# Autodesk Inventor assembly: Backpack
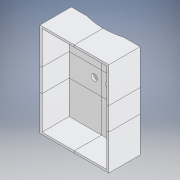
[picture p0: Inventor's stored thumbnail of the model, 180x180]
Saved by Autodesk Inventor 2017 SP1 (Build 210196100, 196)
## iProperties
Created: 2017-09-05
Part Number: Backpack
Document SubType Name: Assembly
Designer: Zach
Author: Zach
## Documents named in this file (8)
- C:\Users\Zach\Documents\GitHub\tr1\src\Body\Chest Assembly\Backpack Assembly\Backpack.iam
- C:\Users\Zach\Documents\GitHub\tr1\src\Body\Chest Assembly\Backpack Assembly\BP001.ipt
- C:\Users\Zach\Documents\GitHub\tr1\src\Body\Chest Assembly\Backpack Assembly\BP002.ipt
- C:\Users\Zach\Documents\GitHub\tr1\src\Body\Chest Assembly\Backpack Assembly\BP003.ipt
- C:\Users\Zach\Documents\GitHub\tr1\src\Body\Chest Assembly\Backpack Assembly\BP004.ipt
- C:\Users\Zach\Documents\GitHub\tr1\src\Body\Chest Assembly\Backpack Assembly\BP005.ipt
- C:\Users\Zach\Documents\GitHub\tr1\src\Body\Chest Assembly\Backpack Assembly\Ethernet Port.ipt
- C:\Users\Zach\Documents\GitHub\tr1\src\Body\Chest Assembly\Backpack Assembly\USB Hub.ipt
## Components (8 placed, 7 different names)
1. BP001:1 — Mate:1, Mate:2, Mate:3, Mate:4, Flush:1, Flush:3, Flush:7, Flush:12, Mate:16, Flush:15, Mate:17, Mate:18, Mate:19, Mate:21
2. BP002:1 — Mate:1, Mate:2, Flush:3, Flush:7, Mate:9, Flush:13, Mate:11, Mate:20
3. BP002:2 — Mate:8, Flush:11, Mate:12, Mate:22
4. BP003:1 — Mate:3, Mate:4, Flush:1, Mate:8, Flush:9, Flush:11, Flush:12, Flush:14
5. BP004:1 — Mate:9, Flush:9, Flush:13, Mate:11, Mate:13, Mate:14
6. BP005:1 — Mate:12, Mate:13, Mate:14
7. Ethernet Port:1 — Flush:14, Mate:18, Mate:19
8. USB Hub:1 — Mate:16, Flush:15, Mate:17
## Relationships (26: Mate 17, Flush 9)
- Mate:1: BP001:1 ↔ BP002:1
- Mate:2: BP001:1 ↔ BP002:1
- Mate:3: BP001:1 ↔ BP003:1
- Mate:4: BP001:1 ↔ BP003:1
- Flush:1: BP001:1 ↔ BP003:1
- Flush:3: BP001:1 ↔ BP002:1
- Flush:7: BP001:1 ↔ BP002:1
- Mate:8: BP002:2 ↔ BP003:1
- Mate:9: BP002:1 ↔ BP004:1
- Flush:9: BP003:1 ↔ BP004:1
- Flush:11: BP002:2 ↔ BP003:1
- Flush:12: BP001:1 ↔ BP003:1
- Flush:13: BP002:1 ↔ BP004:1
- Mate:11: BP002:1 ↔ BP004:1
- Mate:12: BP002:2 ↔ BP005:1
- Mate:13: BP004:1 ↔ BP005:1
- Mate:14: BP004:1 ↔ BP005:1
- Flush:14: BP003:1 ↔ Ethernet Port:1
- Mate:16: BP001:1 ↔ USB Hub:1
- Flush:15: BP001:1 ↔ USB Hub:1
- Mate:17: BP001:1 ↔ USB Hub:1
- Mate:18: BP001:1 ↔ Ethernet Port:1
- Mate:19: BP001:1 ↔ Ethernet Port:1
- Mate:20: BP002:1
- Mate:21: BP001:1
- Mate:22: BP002:2
